# Autodesk Inventor assembly: Recessed Wheels V1.0
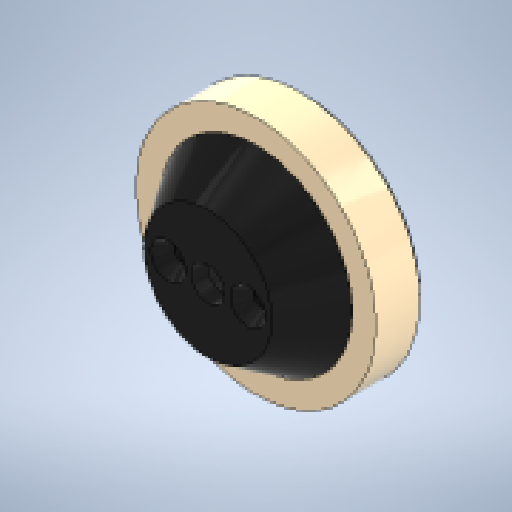
[picture p0: Inventor's stored thumbnail of the model, 512x512]
Saved by Autodesk Inventor 2023.4 (Build 274418000, 418)
## iProperties
Created: 2023-02-06
Part Number: Recessed Wheels V1.0
Document SubType Name: Assembly
Designer: Nathan Cai
Mass: 20.9781 g
Surface Area: 107.263 cm^2
Volume: 17.5686 cm^3
Density: 1.19407 g/cm^3
Author: Nathan Cai
## Documents named in this file (3)
- E:\Documents\Inventor\Shin Impact V1.0\Custom Wheel V1.0\Recessed Wheels V1.0.iam
- E:\Documents\Inventor\Shin Impact V1.0\Custom Wheel V1.0\Tire Hub.ipt
- E:\Documents\Inventor\Shin Impact V1.0\Custom Wheel V1.0\Tire.ipt
## Components (2 placed, 2 different names)
1. Tire Hub:1 — Mate:4, Mate:5
2. Tire:1 — Mate:4, Mate:5
## Relationships (2: Mate 2)
- Mate:4: Tire Hub:1 ↔ Tire:1
- Mate:5: Tire Hub:1 ↔ Tire:1
